# Autodesk Inventor assembly: RightArm
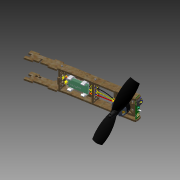
[picture p0: Inventor's stored thumbnail of the model, 180x180]
Saved by Autodesk Inventor 2012 (Build 160160000, 160)
## iProperties
Created: 2014-07-20
Part Number: RightArm
Document SubType Name: Assembly
Designer: Anon
Author: Anon
## Documents named in this file (12)
- D:\Dropbox\Courses\GP\Inventor\dronestructure\RightArm.iam
- D:\Dropbox\Courses\GP\Inventor\dronestructure\MotorCableHolder.ipt
- D:\Dropbox\Courses\GP\Inventor\dronestructure\ESCcableHolder.ipt
- D:\Dropbox\Courses\GP\Inventor\dronestructure\ArmOutside.ipt
- C:\Users\Anon\Documents\Inventor\Content Center Files\R2012\en-US\ISO 4032(2)\ISO 4032 - M2,5ISO.ipt
- C:\Users\Anon\Documents\Inventor\Content Center Files\R2012\en-US\ISO 1207(1)\ISO 1207 - M2,5 x 14DIN EN ISO.ipt
- D:\Dropbox\Courses\GP\Inventor\dronestructure\electronics\afroesc\escassembly.iam
- D:\Dropbox\Courses\GP\Inventor\dronestructure\motor\motormounted.iam
- D:\Dropbox\Courses\GP\Inventor\dronestructure\LeftArm\AIP\Cable and Harness\LeftArm.MotorCables.iam
- D:\Dropbox\Courses\GP\Inventor\dronestructure\electronics\wingleds\wingledpcb\WingLeds.iam
- D:\Dropbox\Courses\GP\Inventor\dronestructure\CrimpSocket.ipt
- D:\Dropbox\Courses\GP\Inventor\dronestructure\ArmInsideHigh.ipt
## Components (21 placed, 11 different names)
1. MotorCableHolder:1 — Flush:8, Flush:9, Mate:66, Mate:72
2. ESCcableHolder:1 — Flush:5, Flush:6, Flush:7, Mate:45, Mate:46, Mate:47, Mate:64, Mate:74
3. ArmOutside:1 — Mate:49, Flush:11, Mate:50, Mate:51, Mate:52, Mate:53, Mate:54, Mate:55, Mate:56
4. ISO 4032 M2,5:1 — Mate:65, Mate:66
5. ISO 4032 M2,5:2 — Mate:73, Mate:74
6. ISO 4032 M2,5:3 — Mate:71, Mate:72
7. ISO 4032 M2,5:4 — Mate:63, Mate:64
8. DIN EN ISO 1207 M2,5 x 14:1 — Mate:61, Mate:62, Mate:63
9. DIN EN ISO 1207 M2,5 x 14:2 — Mate:58, Mate:60, Mate:65
10. DIN EN ISO 1207 M2,5 x 14:3 — Mate:51, Mate:52, Mate:69
11. DIN EN ISO 1207 M2,5 x 14:4 — Mate:55, Mate:56, Mate:73
12. ESC [sub-assembly] — Mate:43, Mate:44, Flush:10
13. Motor [sub-assembly] — Mate:40, Mate:41, Mate:42, Mate:49, Flush:11, Mate:50, Mate:68, Mate:70
14. LeftArm.MotorCables [sub-assembly]
15. DIN EN ISO 1207 M2,5 x 14:5 — Mate:53, Mate:54, Mate:71
16. DIN EN ISO 1207 M2,5 x 14:6 — Mate:57, Mate:59, Mate:67
17. ISO 4032 M2,5:5 — Mate:67, Mate:68
18. ISO 4032 M2,5:6 — Mate:69, Mate:70
19. WingLEDs [sub-assembly]
20. CrimpSocket:1 — Flush:5, Flush:6, Flush:7
21. ArmInsideHigh:1 — Mate:40, Mate:41, Mate:42, Flush:8, Flush:9, Mate:43, Mate:44, Flush:10, Mate:45, Mate:46, Mate:47, Mate:57, Mate:58, Mate:59, Mate:60, Mate:61, Mate:62
## Relationships (41: Mate 34, Flush 7)
- Flush:5: ESCcableHolder:1 ↔ CrimpSocket:1
- Flush:6: ESCcableHolder:1 ↔ CrimpSocket:1
- Flush:7: ESCcableHolder:1 ↔ CrimpSocket:1
- Mate:40: Motor ↔ ArmInsideHigh:1
- Mate:41: Motor ↔ ArmInsideHigh:1
- Mate:42: Motor ↔ ArmInsideHigh:1
- Flush:8: MotorCableHolder:1 ↔ ArmInsideHigh:1
- Flush:9: MotorCableHolder:1 ↔ ArmInsideHigh:1
- Mate:43: ESC ↔ ArmInsideHigh:1
- Mate:44: ESC ↔ ArmInsideHigh:1
- Flush:10: ESC ↔ ArmInsideHigh:1
- Mate:45: ESCcableHolder:1 ↔ ArmInsideHigh:1
- Mate:46: ESCcableHolder:1 ↔ ArmInsideHigh:1
- Mate:47: ESCcableHolder:1 ↔ ArmInsideHigh:1
- Mate:49: ArmOutside:1 ↔ Motor
- Flush:11: ArmOutside:1 ↔ Motor
- Mate:50: ArmOutside:1 ↔ Motor
- Mate:51: ArmOutside:1 ↔ DIN EN ISO 1207 M2,5 x 14:3
- Mate:52: ArmOutside:1 ↔ DIN EN ISO 1207 M2,5 x 14:3
- Mate:53: ArmOutside:1 ↔ DIN EN ISO 1207 M2,5 x 14:5
- Mate:54: ArmOutside:1 ↔ DIN EN ISO 1207 M2,5 x 14:5
- Mate:55: ArmOutside:1 ↔ DIN EN ISO 1207 M2,5 x 14:4
- Mate:56: ArmOutside:1 ↔ DIN EN ISO 1207 M2,5 x 14:4
- Mate:57: DIN EN ISO 1207 M2,5 x 14:6 ↔ ArmInsideHigh:1
- Mate:58: DIN EN ISO 1207 M2,5 x 14:2 ↔ ArmInsideHigh:1
- Mate:59: DIN EN ISO 1207 M2,5 x 14:6 ↔ ArmInsideHigh:1
- Mate:60: DIN EN ISO 1207 M2,5 x 14:2 ↔ ArmInsideHigh:1
- Mate:61: DIN EN ISO 1207 M2,5 x 14:1 ↔ ArmInsideHigh:1
- Mate:62: DIN EN ISO 1207 M2,5 x 14:1 ↔ ArmInsideHigh:1
- Mate:63: ISO 4032 M2,5:4 ↔ DIN EN ISO 1207 M2,5 x 14:1
- Mate:64: ESCcableHolder:1 ↔ ISO 4032 M2,5:4
- Mate:65: ISO 4032 M2,5:1 ↔ DIN EN ISO 1207 M2,5 x 14:2
- Mate:66: MotorCableHolder:1 ↔ ISO 4032 M2,5:1
- Mate:67: DIN EN ISO 1207 M2,5 x 14:6 ↔ ISO 4032 M2,5:5
- Mate:68: Motor ↔ ISO 4032 M2,5:5
- Mate:69: DIN EN ISO 1207 M2,5 x 14:3 ↔ ISO 4032 M2,5:6
- Mate:70: Motor ↔ ISO 4032 M2,5:6
- Mate:71: ISO 4032 M2,5:3 ↔ DIN EN ISO 1207 M2,5 x 14:5
- Mate:72: MotorCableHolder:1 ↔ ISO 4032 M2,5:3
- Mate:73: ISO 4032 M2,5:2 ↔ DIN EN ISO 1207 M2,5 x 14:4
- Mate:74: ESCcableHolder:1 ↔ ISO 4032 M2,5:2
